# Autodesk Inventor assembly: sessao_07_04_999_001
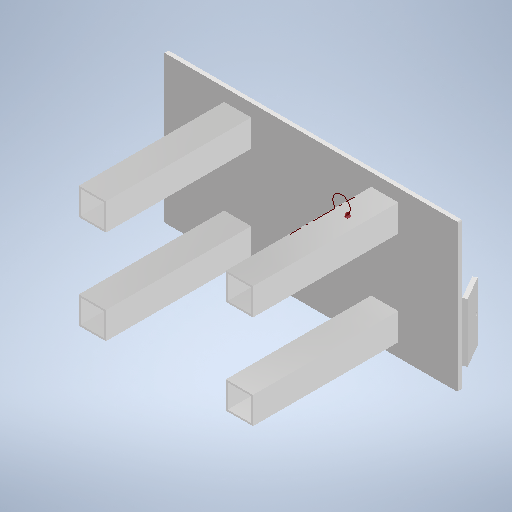
[picture p0: Inventor's stored thumbnail of the model, 512x512]
Saved by Autodesk Inventor 2026 (Build 300175000, 175)
## iProperties
Created: 2025-04-07
Part Number: sessao_07_04_999_001
Document SubType Name: Assembly
Designer: Carlos Dias
Author: Carlos Dias
## Documents named in this file (5)
- C:\Users\Carlos Dias\Documents\Formação-TEARCI\UFCDs\5134 - Robótica _ Fundamentos\Material De Apoio\Sessao_04_04\sessao_07_04_999_001.iam
- C:\Users\Carlos Dias\Documents\Formação-TEARCI\UFCDs\5134 - Robótica _ Fundamentos\Material De Apoio\Sessao_04_04\sessao_07_04_001_001.ipt
- C:\Users\Carlos Dias\Documents\Formação-TEARCI\UFCDs\5134 - Robótica _ Fundamentos\Material De Apoio\Sessao_04_04\sessao_07_04_002_001.ipt
- C:\Users\Carlos Dias\Documents\Formação-TEARCI\UFCDs\5134 - Robótica _ Fundamentos\Material De Apoio\Sessao_04_04\sessao_07_04_003_001.ipt
- C:\Users\Carlos Dias\Documents\Formação-TEARCI\UFCDs\5134 - Robótica _ Fundamentos\Material De Apoio\Sessao_04_04\sessao_07_04_004_001.ipt
## Components (7 placed, 4 different names)
1. sessao_07_04_001_001:1 — Flush:1, Flush:5, Flush:6, Flush:7, Symmetry:1, Symmetry:2, Mate:1, Mate:4
2. sessao_07_04_001_001:2 — Flush:2, Flush:5, Symmetry:1, Mate:2
3. sessao_07_04_001_001:3 — Flush:3, Symmetry:2, Mate:1, Flush:8
4. sessao_07_04_001_001:4 — Flush:4, Flush:8, Mate:2
5. sessao_07_04_002_001:1 — Flush:10, Mate:3, Mate:4, Tangent:1, Mate:6, Flush:11, Angle:1
6. sessao_07_04_004_001:1 — Mate:5, Tangent:1
7. sessao_07_04_003_001:1 — Mate:6, Flush:11, Angle:1
## Relationships (20: Flush 10, Mate 6, Symmetry 2, Tangent 1, Angle 1)
- Flush:1: sessao_07_04_001_001:1
- Flush:2: sessao_07_04_001_001:2
- Flush:3: sessao_07_04_001_001:3
- Flush:4: sessao_07_04_001_001:4
- Flush:5: sessao_07_04_001_001:1 ↔ sessao_07_04_001_001:2
- Flush:6 (125 mm): sessao_07_04_001_001:1
- Flush:7 (-80 mm): sessao_07_04_001_001:1
- Symmetry:1: sessao_07_04_001_001:1 ↔ sessao_07_04_001_001:2
- Symmetry:2: sessao_07_04_001_001:1 ↔ sessao_07_04_001_001:3
- Mate:1: sessao_07_04_001_001:1 ↔ sessao_07_04_001_001:3
- Flush:8: sessao_07_04_001_001:3 ↔ sessao_07_04_001_001:4
- Mate:2: sessao_07_04_001_001:2 ↔ sessao_07_04_001_001:4
- Flush:10: sessao_07_04_002_001:1
- Mate:3: sessao_07_04_002_001:1
- Mate:4: sessao_07_04_001_001:1 ↔ sessao_07_04_002_001:1
- Mate:5: sessao_07_04_004_001:1
- Tangent:1: sessao_07_04_002_001:1 ↔ sessao_07_04_004_001:1
- Mate:6: sessao_07_04_002_001:1 ↔ sessao_07_04_003_001:1
- Flush:11 (35 mm): sessao_07_04_002_001:1 ↔ sessao_07_04_003_001:1
- Angle:1 (-120 deg): sessao_07_04_002_001:1 ↔ sessao_07_04_003_001:1
